# Autodesk Inventor assembly: dlon
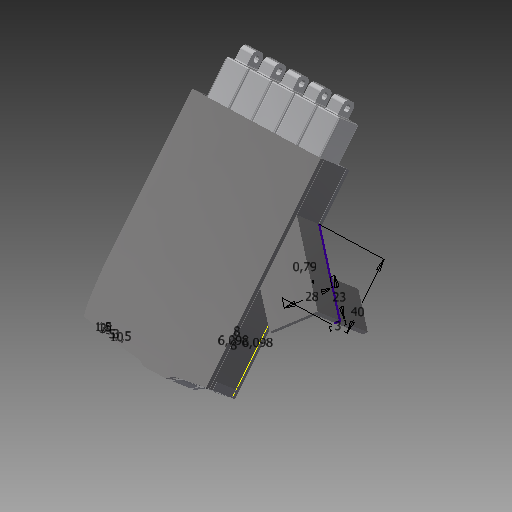
[picture p0: Inventor's stored thumbnail of the model, 512x512]
Saved by Autodesk Inventor 2019 (Build 230136000, 136)
## iProperties
Created: 2019-11-29
Part Number: dlon
Material: Ogólny
Document SubType Name: Assembly
Designer: wojta
Author: wojta
## Documents named in this file (12)
- C:\Users\wojta\Desktop\rekav2\dlon\dlon.iam
- C:\Users\wojta\Desktop\rekav2\dlon\boki.ipt
- C:\Users\wojta\Desktop\rekav2\dlon\pokrywa.ipt
- C:\Users\wojta\Desktop\rekav2\dlon\przod_palce.ipt
- C:\Users\wojta\Desktop\rekav2\dlon\wewnetrzna czec.ipt
- C:\Users\wojta\Desktop\rekav2\serwo\Body serwo.ipt
- C:\Users\wojta\Desktop\rekav2\dlon\podporka.ipt
- C:\Users\wojta\Desktop\rekav2\dlon\Pullie.ipt
- C:\Users\wojta\Desktop\rekav2\dlon\podpora_kciuk.ipt
- C:\Users\wojta\Desktop\rekav2\dlon\Pulley_small.ipt
- C:\Users\wojta\Desktop\rekav2\dlon\belka.ipt
- C:\Users\wojta\Desktop\rekav2\dlon\lozysko.ipt
## Components (67 placed, 11 different names)
1. boki:1 — Sztywne:2, Sztywne:3, Zestawiający:15, Kąt:1, Zestawiający:66, Zestawiający:67, Zestawiający:73, Zestawiający:77, Zestawiający:78, Zestawiający:79
2. pokrywa:1 — Sztywne:3
3. przod_palce:1 — Sztywne:1, Sztywne:2, Zestawiający:72, Styczny:1, Zestawiający:74, Styczny:2, Zestawiający:75, Styczny:3, Zestawiający:76, Styczny:4
4. wewnetrzna czec:1 — Sztywne:1, Zestawiający:16, Zestawiający:19, Zestawiający:22, Zestawiający:24, Zestawiający:60, Zestawiający:61, Zestawiający:62, Zestawiający:63
5. podporka:1 — Zestawiający:16, Zestawiający:17, Zestawiający:18, Zestawiający:28, Zestawiający:32, Zestawiający:38, Zestawiający:39
6. Body serwo:1 — Zestawiający:13, Zestawiający:14, Zestawiający:15, Zestawiający:17, Zestawiający:18, Zestawiający:60, Zestawiający:61
7. Body serwo:2 — Zestawiający:7, Zestawiający:10, Zestawiający:13, Zestawiający:14
8. Body serwo:3 — Zestawiający:8, Zestawiający:12, Zestawiający:23, Zestawiający:26
9. Body serwo:4 — Zestawiający:8, Zestawiający:9, Zestawiający:11, Zestawiający:12
10. Body serwo:5 — Zestawiający:7, Zestawiający:9, Zestawiający:10, Zestawiający:11, Zestawiający:20, Zestawiający:21, Zestawiający:25, Zestawiający:27
11. podporka:2 — Zestawiający:19, Zestawiający:20, Zestawiający:21, Zestawiający:31, Zestawiający:34
12. podporka:3 — Zestawiający:22, Zestawiający:23, Zestawiający:26, Zestawiający:30, Zestawiający:35, Zestawiający:36, Zestawiający:37
13. podporka:4 — Zestawiający:24, Zestawiający:25, Zestawiający:27, Zestawiający:40, Zestawiający:41
14. Pullie:1 — Zestawiający:28, Zestawiający:32
15. Pullie:2 — Zestawiający:31, Zestawiający:34
16. Pullie:3 — Zestawiający:30, Zestawiający:35
17. Pullie:4 — Zestawiający:38, Zestawiający:39
18. Pullie:6 — Zestawiający:36, Zestawiający:37
19. Pullie:7 — Zestawiający:40, Zestawiający:41
20. podpora_kciuk:1 — Zestawiający:63, Zestawiający:64, Zestawiający:65, Zestawiający:66, Zestawiający:69, Zestawiający:71
21. podpora_kciuk:2 — Zestawiający:62, Zestawiający:64, Zestawiający:65, Kąt:1, Zestawiający:67, Zestawiający:68, Zestawiający:70
22. Pulley_small:1 — Zestawiający:69, Zestawiający:71
23. Pulley_small:2 — Zestawiający:68, Zestawiający:70
24. belka:1 — Zestawiający:72, Zestawiający:73, Styczny:1, Zestawiający:80, Zestawiający:81, Zestawiający:82, Zestawiający:83, Zestawiający:84, Zestawiający:85, Zestawiający:86, Zestawiający:87, Zestawiający:88, Zestawiający:89, Równoległy:1, Równoległy:2, Równoległy:3, Równoległy:4, Równoległy:5, Równoległy:6, Równoległy:7, Równoległy:8, Równoległy:9, Równoległy:10, Równoległy:11
25. belka:2 — Zestawiający:74, Styczny:2, Zestawiający:77, Zestawiający:110, Zestawiający:111, Zestawiający:112, Zestawiający:113, Zestawiający:114, Zestawiający:115, Zestawiający:116, Zestawiający:117, Zestawiający:118, Zestawiający:119, Równoległy:32, Równoległy:33, Równoległy:34, Równoległy:35, Równoległy:36, Równoległy:37, Równoległy:38, Równoległy:39, Równoległy:40, Równoległy:41
26. belka:3 — Zestawiający:75, Styczny:3, Zestawiający:78, Zestawiający:100, Zestawiający:101, Zestawiający:102, Zestawiający:103, Zestawiający:104, Zestawiający:105, Zestawiający:106, Zestawiający:107, Zestawiający:108, Zestawiający:109, Równoległy:22, Równoległy:23, Równoległy:24, Równoległy:25, Równoległy:26, Równoległy:27, Równoległy:28, Równoległy:29, Równoległy:30, Równoległy:31
27. belka:4 — Zestawiający:76, Styczny:4, Zestawiający:79, Zestawiający:90, Zestawiający:91, Zestawiający:92, Zestawiający:93, Zestawiający:94, Zestawiający:95, Zestawiający:96, Zestawiający:97, Zestawiający:98, Zestawiający:99, Równoległy:12, Równoległy:13, Równoległy:14, Równoległy:15, Równoległy:16, Równoległy:17, Równoległy:18, Równoległy:19, Równoległy:20, Równoległy:21
28. lozysko:1 — Zestawiający:84, Równoległy:6
29. lozysko:2 — Zestawiający:94, Równoległy:21
30. lozysko:3 — Zestawiający:104, Równoległy:24
31. lozysko:4 — Zestawiający:103, Równoległy:25
32. lozysko:5 — Zestawiający:85, Równoległy:5
33. lozysko:6 — Zestawiający:93, Równoległy:18
34. lozysko:7 — Zestawiający:101, Równoległy:23
35. lozysko:8 — Zestawiający:99, Równoległy:12
36. lozysko:9 — Zestawiający:81, Równoległy:9
37. lozysko:10 — Zestawiający:89, Równoległy:3
38. lozysko:11 — Zestawiający:100, Równoległy:22
39. lozysko:12 — Zestawiający:102, Równoległy:26
40. lozysko:13 — Zestawiający:83, Równoległy:7
41. lozysko:14 — Zestawiający:92, Równoległy:17
42. lozysko:15 — Zestawiający:111, Równoległy:39
43. lozysko:16 — Zestawiający:112, Równoległy:38
44. lozysko:17 — Zestawiający:82, Równoległy:8
45. lozysko:18 — Zestawiający:91, Równoległy:19
46. lozysko:19 — Zestawiający:110, Równoległy:40
47. lozysko:20 — Zestawiający:113, Równoległy:37
48. lozysko:21 — Zestawiający:80, Równoległy:10, Równoległy:11
49. lozysko:22 — Zestawiający:88, Równoległy:2
50. lozysko:23 — Zestawiający:107, Równoległy:29
51. lozysko:24 — Zestawiający:108, Równoległy:30
52. lozysko:25 — Zestawiający:90, Równoległy:20
53. lozysko:26 — Zestawiający:106, Równoległy:28
54. lozysko:27 — Zestawiający:114, Równoległy:36
55. lozysko:28 — Zestawiający:117, Równoległy:32
56. lozysko:29 — Zestawiający:86, Równoległy:1
57. lozysko:30 — Zestawiający:105, Równoległy:27
58. lozysko:31 — Zestawiający:118, Równoległy:34
59. lozysko:32 — Zestawiający:115, Równoległy:41
60. lozysko:33 — Zestawiający:87, Równoległy:4
61. lozysko:34 — Zestawiający:97, Równoległy:14
62. lozysko:35 — Zestawiający:116, Równoległy:35
63. lozysko:36 — Zestawiający:109, Równoległy:31
64. lozysko:37 — Zestawiający:98, Równoległy:13
65. lozysko:38 — Zestawiający:119, Równoległy:33
66. lozysko:39 — Zestawiający:95, Równoległy:16
67. lozysko:40 — Zestawiający:96, Równoległy:15
## Relationships (142: Mate 93, Flush 41, Tangent 4, WeldJoint 3, Angle 1)
- Sztywne:1 [WeldJoint]: przod_palce:1 ↔ wewnetrzna czec:1
- Sztywne:2 [WeldJoint]: boki:1 ↔ przod_palce:1
- Sztywne:3 [WeldJoint]: boki:1 ↔ pokrywa:1
- Zestawiający:7 [Mate]: Body serwo:2 ↔ Body serwo:5
- Zestawiający:8 [Mate]: Body serwo:3 ↔ Body serwo:4
- Zestawiający:9 [Mate]: Body serwo:4 ↔ Body serwo:5
- Zestawiający:10 [Mate]: Body serwo:2 ↔ Body serwo:5
- Zestawiający:11 [Mate]: Body serwo:4 ↔ Body serwo:5
- Zestawiający:12 [Mate]: Body serwo:3 ↔ Body serwo:4
- Zestawiający:13 [Mate]: Body serwo:1 ↔ Body serwo:2
- Zestawiający:14 [Mate]: Body serwo:1 ↔ Body serwo:2
- Zestawiający:15 [Mate]: boki:1 ↔ Body serwo:1
- Zestawiający:16 [Mate]: wewnetrzna czec:1 ↔ podporka:1
- Zestawiający:17 [Mate] (-0.5 mm): podporka:1 ↔ Body serwo:1
- Zestawiający:18 [Mate] (2.5 mm): podporka:1 ↔ Body serwo:1
- Zestawiający:19 [Mate]: wewnetrzna czec:1 ↔ podporka:2
- Zestawiający:20 [Mate] (-0.5 mm): Body serwo:5 ↔ podporka:2
- Zestawiający:21 [Mate] (2.5 mm): Body serwo:5 ↔ podporka:2
- Zestawiający:22 [Mate]: wewnetrzna czec:1 ↔ podporka:3
- Zestawiający:23 [Mate] (-0.5 mm): Body serwo:3 ↔ podporka:3
- Zestawiający:24 [Mate]: wewnetrzna czec:1 ↔ podporka:4
- Zestawiający:25 [Mate]: Body serwo:5 ↔ podporka:4
- Zestawiający:26 [Mate] (2.5 mm): Body serwo:3 ↔ podporka:3
- Zestawiający:27 [Mate] (2.5 mm): Body serwo:5 ↔ podporka:4
- Zestawiający:28 [Mate]: podporka:1 ↔ Pullie:1
- Zestawiający:30 [Mate]: podporka:3 ↔ Pullie:3
- Zestawiający:31 [Mate]: podporka:2 ↔ Pullie:2
- Zestawiający:32 [Mate]: podporka:1 ↔ Pullie:1
- Zestawiający:34 [Mate]: podporka:2 ↔ Pullie:2
- Zestawiający:35 [Mate]: podporka:3 ↔ Pullie:3
- Zestawiający:36 [Mate]: podporka:3 ↔ Pullie:6
- Zestawiający:37 [Mate]: podporka:3 ↔ Pullie:6
- Zestawiający:38 [Mate]: podporka:1 ↔ Pullie:4
- Zestawiający:39 [Mate]: podporka:1 ↔ Pullie:4
- Zestawiający:40 [Mate]: podporka:4 ↔ Pullie:7
- Zestawiający:41 [Mate]: podporka:4 ↔ Pullie:7
- Zestawiający:60 [Mate]: wewnetrzna czec:1 ↔ Body serwo:1
- Zestawiający:61 [Mate]: wewnetrzna czec:1 ↔ Body serwo:1
- Zestawiający:62 [Mate]: wewnetrzna czec:1 ↔ podpora_kciuk:2
- Zestawiający:63 [Mate]: wewnetrzna czec:1 ↔ podpora_kciuk:1
- Zestawiający:64 [Mate] (6 mm): podpora_kciuk:1 ↔ podpora_kciuk:2
- Zestawiający:65 [Mate]: podpora_kciuk:1 ↔ podpora_kciuk:2
- Kąt:1 [Angle] (90 deg): boki:1 ↔ podpora_kciuk:2
- Zestawiający:66 [Mate] (-8.5 mm): boki:1 ↔ podpora_kciuk:1
- Zestawiający:67 [Mate] (49 mm): boki:1 ↔ podpora_kciuk:2
- Zestawiający:68 [Mate]: podpora_kciuk:2 ↔ Pulley_small:2
- Zestawiający:69 [Mate]: podpora_kciuk:1 ↔ Pulley_small:1
- Zestawiający:70 [Mate]: podpora_kciuk:2 ↔ Pulley_small:2
- Zestawiający:71 [Mate]: podpora_kciuk:1 ↔ Pulley_small:1
- Zestawiający:72 [Mate]: przod_palce:1 ↔ belka:1
- Zestawiający:73 [Mate]: boki:1 ↔ belka:1
- Styczny:1 [Tangent]: przod_palce:1 ↔ belka:1
- Zestawiający:74 [Mate]: przod_palce:1 ↔ belka:2
- Styczny:2 [Tangent]: przod_palce:1 ↔ belka:2
- Zestawiający:75 [Mate]: przod_palce:1 ↔ belka:3
- Styczny:3 [Tangent]: przod_palce:1 ↔ belka:3
- Zestawiający:76 [Mate]: przod_palce:1 ↔ belka:4
- Styczny:4 [Tangent]: przod_palce:1 ↔ belka:4
- Zestawiający:77 [Mate]: boki:1 ↔ belka:2
- Zestawiający:78 [Mate]: boki:1 ↔ belka:3
- Zestawiający:79 [Mate]: boki:1 ↔ belka:4
- Zestawiający:80 [Mate]: belka:1 ↔ lozysko:21
- Zestawiający:81 [Mate]: belka:1 ↔ lozysko:9
- Zestawiający:82 [Mate]: belka:1 ↔ lozysko:17
- Zestawiający:83 [Mate]: belka:1 ↔ lozysko:13
- Zestawiający:84 [Mate]: belka:1 ↔ lozysko:1
- Zestawiający:85 [Mate]: belka:1 ↔ lozysko:5
- Zestawiający:86 [Mate]: belka:1 ↔ lozysko:29
- Zestawiający:87 [Mate]: belka:1 ↔ lozysko:33
- Zestawiający:88 [Mate]: belka:1 ↔ lozysko:22
- Zestawiający:89 [Mate]: belka:1 ↔ lozysko:10
- Równoległy:1 [Flush]: belka:1 ↔ lozysko:29
- Równoległy:2 [Flush]: belka:1 ↔ lozysko:22
- Równoległy:3 [Flush]: belka:1 ↔ lozysko:10
- Równoległy:4 [Flush]: belka:1 ↔ lozysko:33
- Równoległy:5 [Flush]: belka:1 ↔ lozysko:5
- Równoległy:6 [Flush]: belka:1 ↔ lozysko:1
- Równoległy:7 [Flush]: belka:1 ↔ lozysko:13
- Równoległy:8 [Flush]: belka:1 ↔ lozysko:17
- Równoległy:9 [Flush]: belka:1 ↔ lozysko:9
- Równoległy:10 [Flush]: belka:1 ↔ lozysko:21
- Równoległy:11 [Flush]: belka:1 ↔ lozysko:21
- Zestawiający:90 [Mate]: belka:4 ↔ lozysko:25
- Zestawiający:91 [Mate]: belka:4 ↔ lozysko:18
- Zestawiający:92 [Mate]: belka:4 ↔ lozysko:14
- Zestawiający:93 [Mate]: belka:4 ↔ lozysko:6
- Zestawiający:94 [Mate]: belka:4 ↔ lozysko:2
- Zestawiający:95 [Mate]: belka:4 ↔ lozysko:39
- Zestawiający:96 [Mate]: belka:4 ↔ lozysko:40
- Zestawiający:97 [Mate]: belka:4 ↔ lozysko:34
- Zestawiający:98 [Mate]: belka:4 ↔ lozysko:37
- Zestawiający:99 [Mate]: belka:4 ↔ lozysko:8
- Równoległy:12 [Flush]: belka:4 ↔ lozysko:8
- Równoległy:13 [Flush]: belka:4 ↔ lozysko:37
- Równoległy:14 [Flush]: belka:4 ↔ lozysko:34
- Równoległy:15 [Flush]: belka:4 ↔ lozysko:40
- Równoległy:16 [Flush]: belka:4 ↔ lozysko:39
- Równoległy:17 [Flush]: belka:4 ↔ lozysko:14
- Równoległy:18 [Flush]: belka:4 ↔ lozysko:6
- Równoległy:19 [Flush]: belka:4 ↔ lozysko:18
- Równoległy:20 [Flush]: belka:4 ↔ lozysko:25
- Równoległy:21 [Flush]: belka:4 ↔ lozysko:2
- Zestawiający:100 [Mate]: belka:3 ↔ lozysko:11
- Zestawiający:101 [Mate]: belka:3 ↔ lozysko:7
- Zestawiający:102 [Mate]: belka:3 ↔ lozysko:12
- Zestawiający:103 [Mate]: belka:3 ↔ lozysko:4
- Zestawiający:104 [Mate]: belka:3 ↔ lozysko:3
- Zestawiający:105 [Mate]: belka:3 ↔ lozysko:30
- Zestawiający:106 [Mate]: belka:3 ↔ lozysko:26
- Zestawiający:107 [Mate]: belka:3 ↔ lozysko:23
- Zestawiający:108 [Mate]: belka:3 ↔ lozysko:24
- Zestawiający:109 [Mate]: belka:3 ↔ lozysko:36
- Równoległy:22 [Flush]: belka:3 ↔ lozysko:11
- Równoległy:23 [Flush]: belka:3 ↔ lozysko:7
- Równoległy:24 [Flush]: belka:3 ↔ lozysko:3
- Równoległy:25 [Flush]: belka:3 ↔ lozysko:4
- Równoległy:26 [Flush]: belka:3 ↔ lozysko:12
- Równoległy:27 [Flush]: belka:3 ↔ lozysko:30
- Równoległy:28 [Flush]: belka:3 ↔ lozysko:26
- Równoległy:29 [Flush]: belka:3 ↔ lozysko:23
- Równoległy:30 [Flush]: belka:3 ↔ lozysko:24
- Równoległy:31 [Flush]: belka:3 ↔ lozysko:36
- Zestawiający:110 [Mate]: belka:2 ↔ lozysko:19
- Zestawiający:111 [Mate]: belka:2 ↔ lozysko:15
- Zestawiający:112 [Mate]: belka:2 ↔ lozysko:16
- Zestawiający:113 [Mate]: belka:2 ↔ lozysko:20
- Zestawiający:114 [Mate]: belka:2 ↔ lozysko:27
- Zestawiający:115 [Mate]: belka:2 ↔ lozysko:32
- Zestawiający:116 [Mate]: belka:2 ↔ lozysko:35
- Zestawiający:117 [Mate]: belka:2 ↔ lozysko:28
- Zestawiający:118 [Mate]: belka:2 ↔ lozysko:31
- Zestawiający:119 [Mate]: belka:2 ↔ lozysko:38
- Równoległy:32 [Flush]: belka:2 ↔ lozysko:28
- Równoległy:33 [Flush]: belka:2 ↔ lozysko:38
- Równoległy:34 [Flush]: belka:2 ↔ lozysko:31
- Równoległy:35 [Flush]: belka:2 ↔ lozysko:35
- Równoległy:36 [Flush]: belka:2 ↔ lozysko:27
- Równoległy:37 [Flush]: belka:2 ↔ lozysko:20
- Równoległy:38 [Flush]: belka:2 ↔ lozysko:16
- Równoległy:39 [Flush]: belka:2 ↔ lozysko:15
- Równoległy:40 [Flush]: belka:2 ↔ lozysko:19
- Równoległy:41 [Flush]: belka:2 ↔ lozysko:32
